# Autodesk Inventor assembly: 可動域確認の間
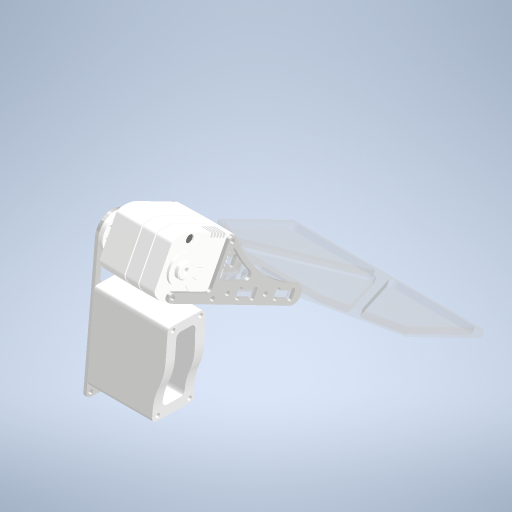
[picture p0: Inventor's stored thumbnail of the model, 512x512]
Saved by Autodesk Inventor 2024 (Build 280153000, 153)
## iProperties
Created: 2024-01-03
Part Number: 可動域確認の間
Document SubType Name: Assembly
Designer: right
Author: right
## Documents named in this file (6)
- C:\Users\right\OneDrive\ドキュメント\Inventor\V2二足Light＿仮\可動域確認の間.iam
- C:\Users\right\OneDrive\ドキュメント\Inventor\V2二足Light＿仮\3204ude.ipt
- C:\Users\right\OneDrive\ドキュメント\Inventor\V2二足Light＿仮\tesaki_arata.iam
- C:\Users\right\OneDrive\ドキュメント\Inventor\V2二足Light＿仮\hera_porika2.ipt
- C:\Users\right\OneDrive\ドキュメント\Inventor\V2二足Light＿仮\02157_SmallDiameterHornB2.ipt
- C:\Users\right\OneDrive\ドキュメント\Inventor\V2二足Light＿仮\3dprintsuzikai.ipt
## Components (5 placed, 5 different names)
1. 3204ude:1 — 挿入:9, 挿入:10, 挿入:13, 挿入:14
2. tesaki_arata:1 [sub-assembly] — 挿入:7, 挿入:8
3. hera_porika2:1 — 挿入:7
4. 02157_SmallDiameterHornB2:2 — 挿入:8, 挿入:9, 挿入:10
5. 3dprintsuzikai:1 — 挿入:13, 挿入:14
## Relationships (7: Insert 7)
- [Insert]: tesaki_arata:1 ↔ hera_porika2:1
- 挿入:7 [Insert]: tesaki_arata:1 ↔ hera_porika2:1
- 挿入:8 [Insert]: tesaki_arata:1 ↔ 02157_SmallDiameterHornB2:2
- 挿入:9 [Insert]: 3204ude:1 ↔ 02157_SmallDiameterHornB2:2
- 挿入:10 [Insert]: 3204ude:1 ↔ 02157_SmallDiameterHornB2:2
- 挿入:13 [Insert]: 3204ude:1 ↔ 3dprintsuzikai:1
- 挿入:14 [Insert]: 3204ude:1 ↔ 3dprintsuzikai:1
